# Autodesk Inventor assembly: launcher.latch
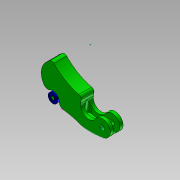
[picture p0: Inventor's stored thumbnail of the model, 180x180]
Saved by Autodesk Inventor 2011 (Build 150239000, 239)
## iProperties
Created: 2011-02-22
Part Number: launcher.latch
Document SubType Name: Assembly
Designer: Casey
Author: Casey
## Documents named in this file (3)
- C:\Users\Casey\Documents\My Dropbox\RockSAT-X 2011 RexSAT\capsule-launcher.design\launcher.latch.iam
- C:\Users\Casey\Documents\My Dropbox\RockSAT-X 2011 RexSAT\capsule-launcher.design\launcher.latch.ipt
- C:\Users\Casey\Documents\My Dropbox\RockSAT-X 2011 RexSAT\capsule-launcher.design\2x6x2.5Bearing.ipt
## Components (3 placed, 2 different names)
1. launcher.latch:1 — Mate:1, Mate:2, Flush:1, Flush:2
2. 2x6x2.5Bearing:1 — Mate:1, Flush:2
3. 2x6x2.5Bearing:2 — Mate:2, Flush:1
## Relationships (4: Mate 2, Flush 2)
- Mate:1: launcher.latch:1 ↔ 2x6x2.5Bearing:1
- Mate:2: launcher.latch:1 ↔ 2x6x2.5Bearing:2
- Flush:1: launcher.latch:1 ↔ 2x6x2.5Bearing:2
- Flush:2: launcher.latch:1 ↔ 2x6x2.5Bearing:1
